# Autodesk Inventor assembly: LMG40-T4
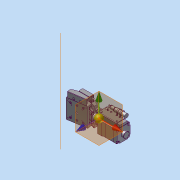
[picture p0: Inventor's stored thumbnail of the model, 180x180]
Saved by Autodesk Inventor 2015 SP1 (Build 190203100, 203)
## iProperties
Created: 2015-02-13
Vendor: ZABER
Document SubType Name: Assembly
Designer: ARNOLDJ
Mass: 359.699 g
Surface Area: 329.157 cm^2
Volume: 73.9979 cm^3
Description: MOTORIZED GONIOMETER STAGE, 40MM RADIUS
Part Number: LMG40-T4
RuleStatus: InUse
AfterDocSave0: file://Part Number Cleaner
DESIGN DEPARTMENT: HHMI: JRC - ID&F
ALTERED ITEM PART NUMBER: N/A
ALTERED ITEM VENDOR: N/A
ALTERED ITEM DESCRIPTION: N/A
Title: LMG40.STEP
Description: STEP AP203
Creation Date: 2010-07-07
Sending System: SolidWorks 2007
Preprocessor: SwSTEP 2.0
Revision Number: 0
## Documents named in this file (3)
- C:\_WORKSPACE\DATA\PROJECTS\MOUSE POSITIONING SYSTEM\MCAD\BALL SETUP\LMG40.iam
- C:\_WORKSPACE\DATA\PROJECTS\MOUSE POSITIONING SYSTEM\MCAD\BALL SETUP\LMG40 Base.ipt
- C:\_WORKSPACE\DATA\PROJECTS\MOUSE POSITIONING SYSTEM\MCAD\BALL SETUP\LMG40 Stage.ipt
## Components (2 placed, 2 different names)
1. LMG40 Base_1 — Flush:1, Mate:1, Mate:2, Angle:1
2. LMG40 Stage_2 — Flush:1, Mate:2, Angle:1
## Relationships (4: Mate 2, Flush 1, Angle 1)
- Flush:1: LMG40 Base_1 ↔ LMG40 Stage_2
- Mate:1: LMG40 Base_1
- Mate:2: LMG40 Base_1 ↔ LMG40 Stage_2
- Angle:1 (0 deg): LMG40 Base_1 ↔ LMG40 Stage_2
